# Autodesk Inventor assembly: ZAxisBed
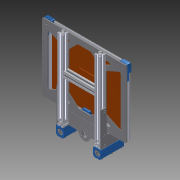
[picture p0: Inventor's stored thumbnail of the model, 180x180]
Saved by Autodesk Inventor 2015 SP1 (Build 190203100, 203)
## iProperties
Created: 2015-01-21
Part Number: ZAxisBed
Document SubType Name: Assembly
Designer: Jack
Mass: 2277.03 g
Surface Area: 6915.31 cm^2
Volume: 775.989 cm^3
Density: 2.93435 g/cm^3
Author: Jack
Title: Bed + Z Carriage
## Documents named in this file (22)
- C:\Users\Jack\ownCloud\Projects\CrossBot\InventorModel\ZAxis\ZAxisBed.iam
- C:\Users\Jack\ownCloud\Projects\CrossBot\InventorModel\Hardware\Bearing\BearingLinear\BearingLinearLMU10.ipt
- C:\Users\Jack\ownCloud\Projects\CrossBot\InventorModel\ZAxis\ZAxisCarriageRight.ipt
- C:\Users\Jack\ownCloud\Projects\CrossBot\InventorModel\ZAxis\ZAxisCarriageLeft.ipt
- C:\Users\Jack\ownCloud\Projects\CrossBot\InventorModel\HeatBed\Ultibots230x290\UltibotsBed230x290.iam
- C:\Users\Jack\ownCloud\Projects\CrossBot\InventorModel\ZAxis\ZAxisFrameVertical.ipt
- C:\Users\Jack\ownCloud\Projects\CrossBot\InventorModel\ZAxis\ZBedSupportExtrusion.ipt
- C:\Users\Jack\ownCloud\Projects\CrossBot\InventorModel\ZAxis\ZBedPlate.ipt
- C:\Users\Jack\ownCloud\Projects\CrossBot\InventorModel\HeatBed\BedClipUltiBots.ipt
- C:\Users\Jack\ownCloud\Projects\CrossBot\InventorModel\HeatBed\BedClipUltiBotsMirrored.ipt
- C:\Users\Jack\ownCloud\Projects\CrossBot\InventorModel\Hardware\Nuts\Nut3.ipt
- C:\Users\Jack\ownCloud\Projects\CrossBot\InventorModel\ZAxis\ZBedSupportLateral.ipt
- C:\Users\Jack\ownCloud\Projects\CrossBot\InventorModel\ZAxis\ZBedSupportPlate.ipt
- C:\Users\Jack\ownCloud\Projects\CrossBot\InventorModel\ZAxis\ZAxisNutMountMetal.ipt
- C:\Users\Jack\ownCloud\Projects\CrossBot\InventorModel\Hardware\Nuts\Nut4.ipt
- C:\Users\Jack\ownCloud\Projects\CrossBot\InventorModel\Hardware\BoltWashers\BoltWasher3\BoltWasher3x24.iam
- C:\Users\Jack\ownCloud\Projects\CrossBot\InventorModel\Hardware\BoltWashers\BoltWasher4\BoltWasher4x10.iam
- C:\Users\Jack\ownCloud\Projects\CrossBot\InventorModel\Hardware\Bolts\FHS\FHS4\FHS4x12.ipt
- C:\Users\Jack\ownCloud\Projects\CrossBot\InventorModel\Hardware\BoltWashers\BoltWasher3\BoltWasher3x16.iam
- C:\Users\Jack\ownCloud\Projects\CrossBot\InventorModel\Hardware\Wahsers\M3Washer.ipt
- C:\Users\Jack\ownCloud\Projects\CrossBot\InventorModel\HeatBed\BedClipUltiBotsMiddle.ipt
- C:\Users\Jack\ownCloud\Projects\CrossBot\InventorModel\Hardware\ZDrive\ZACMENut.ipt
## Components (72 placed, 21 different names)
1. BedClipUltiBotsMiddle:1 — Mate:196, Mate:197, Angle:25
2. BedClipUltiBotsMirrored:1
3. BedClipUltiBots:1
4. ZBedPlate:1 — Mate:76, Flush:23, Flush:34, Flush:35, Mate:196, Mate:197
5. UltibotsBed230x290:1 [sub-assembly] — Angle:25
6. ZAxisFrameVertical:1 — Mate:75, Flush:18, Flush:19, Mate:82, Flush:28, Flush:29, Mate:86, Mate:90, Mate:116, Mate:117, Mate:118, Angle:11, Angle:12, Angle:13, Mate:156, Mate:157, Mate:158, Mate:173, Mate:174, Angle:18, Angle:19
7. ZAxisFrameVertical:2 — Mate:74, Flush:17, Flush:20, Mate:78, Mate:80, Flush:26, Flush:30, Mate:84, Mate:113, Mate:115, Angle:14, Angle:15, Mate:153, Mate:154, Mate:155, Mate:163, Mate:164, Angle:16, Angle:17, Mate:176, Mate:178, Angle:24, Mate:180
8. ZBedSupportExtrusion:1 — Mate:74, Flush:17, Flush:20, Flush:22, Flush:32, Flush:34, Mate:165, Mate:166, Angle:22, Angle:23
9. ZBedSupportExtrusion:2 — Mate:75, Flush:18, Flush:19, Mate:76, Mate:77, Flush:23, Mate:83, Flush:31, Flush:33, Mate:88, Mate:171, Mate:172, Angle:20, Angle:21
10. ZBedSupportLateral:1 — Mate:77, Flush:22, Mate:83, Flush:31, Flush:35
11. ZAxisNutMountMetal:1 — Mate:88, Mate:89, Mate:90, Mate:192, Mate:193, Mate:195, Mate:210, Mate:211, Mate:212, Mate:213, Mate:214, Mate:215, Mate:216
12. ZACMENut:2 — Mate:215, Mate:216, Mate:217, Mate:218, Mate:219, Mate:220, Mate:221
13. BoltWasher3x16:1 [sub-assembly] — Mate:194, Mate:198, Mate:213, Mate:218
14. BoltWasher3x16:3 [sub-assembly] — Mate:190, Mate:199, Mate:212, Mate:219
15. BoltWasher3x16:2 [sub-assembly] — Mate:191, Mate:200, Mate:214, Mate:217, Mate:220
16. BoltWasher3x16:4 [sub-assembly] — Mate:210, Mate:221
17. Nut3:10
18. M3Washer:4 — Mate:211
19. M3Washer:1 — Mate:190, Mate:193, Mate:202
20. Nut3:8 — Mate:199, Mate:202
21. Nut3:9 — Mate:198, Mate:203
22. M3Washer:3 — Mate:194, Mate:195, Mate:203
23. Nut3:7 — Mate:200, Mate:201
24. M3Washer:2 — Mate:191, Mate:192, Mate:201
25. Nut4:3 — Mate:116, Angle:13, Mate:183
26. Nut4:2 — Mate:117, Angle:12, Mate:182
27. Nut4:1 — Mate:118, Angle:11, Mate:181
28. FHS4x12:1 — Mate:152, Mate:156, Mate:183
29. FHS4x12:2 — Mate:151, Mate:157, Mate:182
30. FHS4x12:3 — Mate:150, Mate:158, Mate:181
31. BearingLinearLMU10:3 — Mate:37, Flush:16
32. BearingLinearLMU10:2 — Mate:42
33. ZAxisCarriageRight:1 — Mate:37, Flush:16, Angle:5, Angle:6, Angle:7, Mate:62, Mate:63, Mate:64, Flush:27, Mate:82, Flush:28, Flush:29, Mate:87, Mate:125, Mate:126, Mate:127, Mate:128, Mate:129, Mate:130, Mate:150, Mate:151, Mate:152
34. Nut4:5 — Mate:115, Angle:14, Mate:175, Mate:176
35. Nut4:6 — Mate:113, Angle:15, Mate:177, Mate:178
36. Nut4:15 — Mate:179, Angle:24, Mate:180
37. FHS4x12:6 — Mate:149, Mate:155, Mate:179
38. FHS4x12:5 — Mate:148, Mate:154, Mate:177
39. FHS4x12:4 — Mate:147, Mate:153, Mate:175
40. ZAxisCarriageLeft:1 — Mate:36, Flush:15, Angle:8, Angle:9, Angle:10, Mate:65, Mate:66, Mate:67, Mate:78, Flush:24, Mate:79, Flush:25, Mate:80, Flush:26, Flush:27, Flush:30, Mate:85, Mate:119, Mate:120, Mate:121, Mate:122, Mate:123, Mate:124, Mate:147, Mate:148, Mate:149
41. BearingLinearLMU10:4 — Mate:36, Flush:15
42. BearingLinearLMU10:1 — Mate:42
43. BoltWasher4x10:2 [sub-assembly] — Mate:133, Mate:134, Mate:160
44. Nut4:10 — Mate:160, Mate:164, Angle:17
45. BoltWasher4x10:1 [sub-assembly] — Mate:131, Mate:132, Mate:159
46. Nut4:7 — Mate:159, Mate:163, Angle:16
47. BoltWasher4x10:3 [sub-assembly] — Mate:135, Mate:136, Mate:161
48. Nut4:8 — Mate:161, Mate:165, Angle:22
49. Nut4:9 — Mate:162, Mate:166, Angle:23
50. BoltWasher4x10:4 [sub-assembly] — Mate:137, Mate:138, Mate:162
51. ZBedSupportPlate:1 — Mate:84, Flush:32, Mate:85, Mate:131, Mate:132, Mate:133, Mate:134, Mate:135, Mate:136, Mate:137, Mate:138
52. BoltWasher4x10:7 [sub-assembly] — Mate:141, Mate:143, Mate:170
53. BoltWasher4x10:8 [sub-assembly] — Mate:140, Mate:144, Mate:169
54. BoltWasher4x10:5 [sub-assembly] — Mate:139, Mate:145, Mate:168
55. Nut4:13 — Mate:168, Mate:173, Angle:19
56. Nut4:12 — Mate:169, Mate:172, Angle:20
57. Nut4:14 — Mate:170, Mate:171, Angle:21
58. Nut4:11 — Mate:167, Mate:174, Angle:18
59. BoltWasher4x10:6 [sub-assembly] — Mate:142, Mate:146, Mate:167
60. ZBedSupportPlate:2 — Mate:86, Mate:87, Flush:33, Mate:89, Mate:139, Mate:140, Mate:141, Mate:142, Mate:143, Mate:144, Mate:145, Mate:146
61. BoltWasher3x24:5 [sub-assembly] — Mate:127, Mate:128
62. Nut3:3 — Angle:7, Mate:64
63. Nut3:1 — Angle:6, Mate:63
64. BoltWasher3x24:4 [sub-assembly] — Mate:126, Mate:129
65. BoltWasher3x24:6 [sub-assembly] — Mate:125, Mate:130
66. Nut3:2 — Angle:5, Mate:62
67. Nut3:6 — Angle:8, Mate:65
68. BoltWasher3x24:2 [sub-assembly] — Mate:119, Mate:124
69. Nut3:5 — Angle:9, Mate:66
70. BoltWasher3x24:3 [sub-assembly] — Mate:120, Mate:123
71. BoltWasher3x24:1 [sub-assembly] — Mate:121, Mate:122
72. Nut3:4 — Angle:10, Mate:67
## Relationships (181: Mate 133, Flush 25, Angle 23)
- [Mate]: ZAxisCarriageLeft:1 ↔ BearingLinearLMU10:1
- [Mate]: BearingLinearLMU10:2 ↔ ZAxisCarriageRight:1
- [Flush]: BearingLinearLMU10:2 ↔ ZAxisCarriageRight:1
- [Flush]: ZAxisCarriageLeft:1 ↔ BearingLinearLMU10:1
- [Flush]: ZAxisCarriageLeft:1 ↔ BearingLinearLMU10:4
- [Flush]: BearingLinearLMU10:3 ↔ ZAxisCarriageRight:1
- [Flush]: ZAxisCarriageRight:1 ↔ ZAxisCarriageLeft:1
- [Mate]: BedClipUltiBotsMirrored:1 ↔ ZBedPlate:1
- [Mate]: BedClipUltiBots:1 ↔ ZBedPlate:1
- [Mate] (2 mm): BedClipUltiBots:1 ↔ ZBedPlate:1
- [Mate] (2 mm): BedClipUltiBotsMirrored:1 ↔ ZBedPlate:1
- [Angle] (0 deg): BedClipUltiBots:1 ↔ ZBedPlate:1
- [Angle] (0 deg): BedClipUltiBotsMirrored:1 ↔ ZBedPlate:1
- [Mate]: BedClipUltiBotsMirrored:1 ↔ UltibotsBed230x290:1
- [Mate]: BedClipUltiBots:1 ↔ UltibotsBed230x290:1
- [Mate]: BedClipUltiBots:1 ↔ UltibotsBed230x290:1
- Mate:36: ZAxisCarriageLeft:1 ↔ BearingLinearLMU10:4
- Flush:15: ZAxisCarriageLeft:1 ↔ BearingLinearLMU10:4
- Mate:37: BearingLinearLMU10:3 ↔ ZAxisCarriageRight:1
- Flush:16: BearingLinearLMU10:3 ↔ ZAxisCarriageRight:1
- Mate:42 (130 mm): BearingLinearLMU10:2 ↔ BearingLinearLMU10:1
- Angle:5 (0 deg): ZAxisCarriageRight:1 ↔ Nut3:2
- Angle:6 (0 deg): ZAxisCarriageRight:1 ↔ Nut3:1
- Angle:7 (0 deg): ZAxisCarriageRight:1 ↔ Nut3:3
- Angle:8 (0 deg): ZAxisCarriageLeft:1 ↔ Nut3:6
- Angle:9 (0 deg): ZAxisCarriageLeft:1 ↔ Nut3:5
- Angle:10 (0 deg): ZAxisCarriageLeft:1 ↔ Nut3:4
- Mate:62: ZAxisCarriageRight:1 ↔ Nut3:2
- Mate:63: ZAxisCarriageRight:1 ↔ Nut3:1
- Mate:64: ZAxisCarriageRight:1 ↔ Nut3:3
- Mate:65: ZAxisCarriageLeft:1 ↔ Nut3:6
- Mate:66: ZAxisCarriageLeft:1 ↔ Nut3:5
- Mate:67: ZAxisCarriageLeft:1 ↔ Nut3:4
- Mate:74: ZAxisFrameVertical:2 ↔ ZBedSupportExtrusion:1
- Flush:17: ZAxisFrameVertical:2 ↔ ZBedSupportExtrusion:1
- Mate:75: ZAxisFrameVertical:1 ↔ ZBedSupportExtrusion:2
- Flush:18: ZAxisFrameVertical:1 ↔ ZBedSupportExtrusion:2
- Flush:19: ZAxisFrameVertical:1 ↔ ZBedSupportExtrusion:2
- Flush:20: ZAxisFrameVertical:2 ↔ ZBedSupportExtrusion:1
- Mate:76: ZBedPlate:1 ↔ ZBedSupportExtrusion:2
- Mate:77: ZBedSupportExtrusion:2 ↔ ZBedSupportLateral:1
- Flush:22: ZBedSupportExtrusion:1 ↔ ZBedSupportLateral:1
- Flush:23 (-73 mm): ZBedPlate:1 ↔ ZBedSupportExtrusion:2
- Mate:78: ZAxisFrameVertical:2 ↔ ZAxisCarriageLeft:1
- Flush:24: ZAxisCarriageLeft:1
- Mate:79: ZAxisCarriageLeft:1
- Flush:25: ZAxisCarriageLeft:1
- Mate:80: ZAxisFrameVertical:2 ↔ ZAxisCarriageLeft:1
- Flush:26 (4 mm): ZAxisFrameVertical:2 ↔ ZAxisCarriageLeft:1
- Flush:27: ZAxisCarriageRight:1 ↔ ZAxisCarriageLeft:1
- Mate:82: ZAxisFrameVertical:1 ↔ ZAxisCarriageRight:1
- Flush:28 (4 mm): ZAxisFrameVertical:1 ↔ ZAxisCarriageRight:1
- Flush:29: ZAxisFrameVertical:1 ↔ ZAxisCarriageRight:1
- Flush:30: ZAxisFrameVertical:2 ↔ ZAxisCarriageLeft:1
- Mate:83: ZBedSupportExtrusion:2 ↔ ZBedSupportLateral:1
- Flush:31: ZBedSupportExtrusion:2 ↔ ZBedSupportLateral:1
- Mate:84: ZAxisFrameVertical:2 ↔ ZBedSupportPlate:1
- Flush:32: ZBedSupportExtrusion:1 ↔ ZBedSupportPlate:1
- Mate:85: ZAxisCarriageLeft:1 ↔ ZBedSupportPlate:1
- Mate:86: ZAxisFrameVertical:1 ↔ ZBedSupportPlate:2
- Mate:87: ZAxisCarriageRight:1 ↔ ZBedSupportPlate:2
- Flush:33: ZBedSupportExtrusion:2 ↔ ZBedSupportPlate:2
- Flush:34: ZBedPlate:1 ↔ ZBedSupportExtrusion:1
- Flush:35 (108.25 mm): ZBedPlate:1 ↔ ZBedSupportLateral:1
- Mate:88: ZBedSupportExtrusion:2 ↔ ZAxisNutMountMetal:1
- Mate:89: ZAxisNutMountMetal:1 ↔ ZBedSupportPlate:2
- Mate:90: ZAxisFrameVertical:1 ↔ ZAxisNutMountMetal:1
- Mate:113: ZAxisFrameVertical:2 ↔ Nut4:6
- Mate:115: ZAxisFrameVertical:2 ↔ Nut4:5
- Mate:116: ZAxisFrameVertical:1 ↔ Nut4:3
- Mate:117: ZAxisFrameVertical:1 ↔ Nut4:2
- Mate:118: ZAxisFrameVertical:1 ↔ Nut4:1
- Angle:11 (0 deg): ZAxisFrameVertical:1 ↔ Nut4:1
- Angle:12 (0 deg): ZAxisFrameVertical:1 ↔ Nut4:2
- Angle:13 (0 deg): ZAxisFrameVertical:1 ↔ Nut4:3
- Angle:14 (0 deg): ZAxisFrameVertical:2 ↔ Nut4:5
- Angle:15 (0 deg): ZAxisFrameVertical:2 ↔ Nut4:6
- Mate:119: ZAxisCarriageLeft:1 ↔ BoltWasher3x24:2
- Mate:120: ZAxisCarriageLeft:1 ↔ BoltWasher3x24:3
- Mate:121: ZAxisCarriageLeft:1 ↔ BoltWasher3x24:1
- Mate:122: ZAxisCarriageLeft:1 ↔ BoltWasher3x24:1
- Mate:123: ZAxisCarriageLeft:1 ↔ BoltWasher3x24:3
- Mate:124: ZAxisCarriageLeft:1 ↔ BoltWasher3x24:2
- Mate:125: ZAxisCarriageRight:1 ↔ BoltWasher3x24:6
- Mate:126: ZAxisCarriageRight:1 ↔ BoltWasher3x24:4
- Mate:127: ZAxisCarriageRight:1 ↔ BoltWasher3x24:5
- Mate:128: ZAxisCarriageRight:1 ↔ BoltWasher3x24:5
- Mate:129: ZAxisCarriageRight:1 ↔ BoltWasher3x24:4
- Mate:130: ZAxisCarriageRight:1 ↔ BoltWasher3x24:6
- Mate:131: BoltWasher4x10:1 ↔ ZBedSupportPlate:1
- Mate:132: BoltWasher4x10:1 ↔ ZBedSupportPlate:1
- Mate:133: BoltWasher4x10:2 ↔ ZBedSupportPlate:1
- Mate:134: BoltWasher4x10:2 ↔ ZBedSupportPlate:1
- Mate:135: BoltWasher4x10:3 ↔ ZBedSupportPlate:1
- Mate:136: BoltWasher4x10:3 ↔ ZBedSupportPlate:1
- Mate:137: BoltWasher4x10:4 ↔ ZBedSupportPlate:1
- Mate:138: BoltWasher4x10:4 ↔ ZBedSupportPlate:1
- Mate:139: BoltWasher4x10:5 ↔ ZBedSupportPlate:2
- Mate:140: BoltWasher4x10:8 ↔ ZBedSupportPlate:2
- Mate:141: BoltWasher4x10:7 ↔ ZBedSupportPlate:2
- Mate:142: BoltWasher4x10:6 ↔ ZBedSupportPlate:2
- Mate:143: BoltWasher4x10:7 ↔ ZBedSupportPlate:2
- Mate:144: BoltWasher4x10:8 ↔ ZBedSupportPlate:2
- Mate:145: BoltWasher4x10:5 ↔ ZBedSupportPlate:2
- Mate:146: BoltWasher4x10:6 ↔ ZBedSupportPlate:2
- Mate:147: FHS4x12:4 ↔ ZAxisCarriageLeft:1
- Mate:148: FHS4x12:5 ↔ ZAxisCarriageLeft:1
- Mate:149: FHS4x12:6 ↔ ZAxisCarriageLeft:1
- Mate:150: FHS4x12:3 ↔ ZAxisCarriageRight:1
- Mate:151: FHS4x12:2 ↔ ZAxisCarriageRight:1
- Mate:152: FHS4x12:1 ↔ ZAxisCarriageRight:1
- Mate:153 (0.5 mm): ZAxisFrameVertical:2 ↔ FHS4x12:4
- Mate:154 (0.5 mm): ZAxisFrameVertical:2 ↔ FHS4x12:5
- Mate:155 (0.5 mm): ZAxisFrameVertical:2 ↔ FHS4x12:6
- Mate:156 (0.5 mm): ZAxisFrameVertical:1 ↔ FHS4x12:1
- Mate:157 (0.5 mm): ZAxisFrameVertical:1 ↔ FHS4x12:2
- Mate:158 (0.5 mm): ZAxisFrameVertical:1 ↔ FHS4x12:3
- Mate:159: BoltWasher4x10:1 ↔ Nut4:7
- Mate:160: BoltWasher4x10:2 ↔ Nut4:10
- Mate:161: BoltWasher4x10:3 ↔ Nut4:8
- Mate:162: Nut4:9 ↔ BoltWasher4x10:4
- Mate:163: ZAxisFrameVertical:2 ↔ Nut4:7
- Mate:164: ZAxisFrameVertical:2 ↔ Nut4:10
- Mate:165: ZBedSupportExtrusion:1 ↔ Nut4:8
- Mate:166: ZBedSupportExtrusion:1 ↔ Nut4:9
- Mate:167: Nut4:11 ↔ BoltWasher4x10:6
- Mate:168: BoltWasher4x10:5 ↔ Nut4:13
- Mate:169: BoltWasher4x10:8 ↔ Nut4:12
- Mate:170: BoltWasher4x10:7 ↔ Nut4:14
- Mate:171: ZBedSupportExtrusion:2 ↔ Nut4:14
- Mate:172: ZBedSupportExtrusion:2 ↔ Nut4:12
- Mate:173: ZAxisFrameVertical:1 ↔ Nut4:13
- Mate:174: ZAxisFrameVertical:1 ↔ Nut4:11
- Angle:16 (0 deg): ZAxisFrameVertical:2 ↔ Nut4:7
- Angle:17 (0 deg): ZAxisFrameVertical:2 ↔ Nut4:10
- Angle:18 (0 deg): ZAxisFrameVertical:1 ↔ Nut4:11
- Angle:19 (0 deg): ZAxisFrameVertical:1 ↔ Nut4:13
- Angle:20 (0 deg): ZBedSupportExtrusion:2 ↔ Nut4:12
- Angle:21 (0 deg): ZBedSupportExtrusion:2 ↔ Nut4:14
- Angle:22 (0 deg): ZBedSupportExtrusion:1 ↔ Nut4:8
- Angle:23 (0 deg): ZBedSupportExtrusion:1 ↔ Nut4:9
- Mate:175: Nut4:5 ↔ FHS4x12:4
- Mate:176: ZAxisFrameVertical:2 ↔ Nut4:5
- Mate:177: Nut4:6 ↔ FHS4x12:5
- Mate:178: ZAxisFrameVertical:2 ↔ Nut4:6
- Mate:179: Nut4:15 ↔ FHS4x12:6
- Angle:24 (0 deg): ZAxisFrameVertical:2 ↔ Nut4:15
- Mate:180: ZAxisFrameVertical:2 ↔ Nut4:15
- Mate:181: Nut4:1 ↔ FHS4x12:3
- Mate:182: Nut4:2 ↔ FHS4x12:2
- Mate:183: Nut4:3 ↔ FHS4x12:1
- Mate:190: BoltWasher3x16:3 ↔ M3Washer:1
- Mate:191: BoltWasher3x16:2 ↔ M3Washer:2
- Mate:192: ZAxisNutMountMetal:1 ↔ M3Washer:2
- Mate:193: ZAxisNutMountMetal:1 ↔ M3Washer:1
- Mate:194: BoltWasher3x16:1 ↔ M3Washer:3
- Mate:195: ZAxisNutMountMetal:1 ↔ M3Washer:3
- Mate:196: BedClipUltiBotsMiddle:1 ↔ ZBedPlate:1
- Mate:197 (2 mm): BedClipUltiBotsMiddle:1 ↔ ZBedPlate:1
- Angle:25 (0 deg): BedClipUltiBotsMiddle:1 ↔ UltibotsBed230x290:1
- Mate:198: BoltWasher3x16:1 ↔ Nut3:9
- Mate:199: BoltWasher3x16:3 ↔ Nut3:8
- Mate:200: BoltWasher3x16:2 ↔ Nut3:7
- Mate:201: Nut3:7 ↔ M3Washer:2
- Mate:202: M3Washer:1 ↔ Nut3:8
- Mate:203: Nut3:9 ↔ M3Washer:3
- [Mate]: BoltWasher3x16:4 ↔ M3Washer:4
- [Mate]: BoltWasher3x16:4 ↔ Nut3:10
- [Mate]: Nut3:10 ↔ M3Washer:4
- Mate:210: ZAxisNutMountMetal:1 ↔ BoltWasher3x16:4
- Mate:211: ZAxisNutMountMetal:1 ↔ M3Washer:4
- Mate:212: ZAxisNutMountMetal:1 ↔ BoltWasher3x16:3
- Mate:213: ZAxisNutMountMetal:1 ↔ BoltWasher3x16:1
- Mate:214: ZAxisNutMountMetal:1 ↔ BoltWasher3x16:2
- Mate:215: ZAxisNutMountMetal:1 ↔ ZACMENut:2
- Mate:216: ZAxisNutMountMetal:1 ↔ ZACMENut:2
- Mate:217: ZACMENut:2 ↔ BoltWasher3x16:2
- Mate:218: ZACMENut:2 ↔ BoltWasher3x16:1
- Mate:219: ZACMENut:2 ↔ BoltWasher3x16:3
- Mate:220: ZACMENut:2 ↔ BoltWasher3x16:2
- Mate:221: ZACMENut:2 ↔ BoltWasher3x16:4
## Named parameters: d373_d360 = 0 mm, d374_d365 = 0 mm, d375_d370 = 0 mm
